# Autodesk Inventor assembly: Chassis and wheels assembly
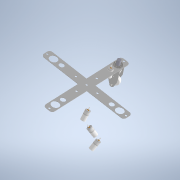
[picture p0: Inventor's stored thumbnail of the model, 180x180]
Saved by Autodesk Inventor 2020 (Build 240168000, 168)
## iProperties
Created: 2022-07-01
Part Number: Chassis and wheels assembly
Document SubType Name: Assembly
Designer: karimi2
Author: karimi2
## Documents named in this file (4)
- C:\Users\karimi2\Documents\PROJECT\Chassis and wheels assembly.iam
- C:\Users\karimi2\Documents\PROJECT\src\chassisPart1.ipt
- C:\Users\karimi2\Documents\PROJECT\src\GearedDCmotor.ipt
- C:\Users\karimi2\Documents\PROJECT\src\Wheel Assembly.iam
## Components (7 placed, 3 different names)
1. chassisPart1:1 — Rigid:1, Rigid:2, Rigid:3
2. chassisPart1:2 — Rigid:1
3. GearedDCmotor:1 — Rigid:2
4. GearedDCmotor:2
5. GearedDCmotor:3
6. GearedDCmotor:4
7. Wheel Assembly:1 [sub-assembly] — Rigid:3
## Relationships (3: WeldJoint 3)
- Rigid:1 [WeldJoint]: chassisPart1:1 ↔ chassisPart1:2
- Rigid:2 [WeldJoint]: chassisPart1:1 ↔ GearedDCmotor:1
- Rigid:3 [WeldJoint] (4.5 mm): chassisPart1:1 ↔ Wheel Assembly:1
